# Autodesk Inventor assembly: SC8UU
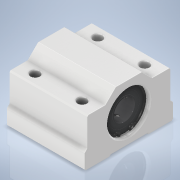
[picture p0: Inventor's stored thumbnail of the model, 180x180]
Saved by Autodesk Inventor 2020.2 (Build 242310000, 310)
## iProperties
Created: 2020-07-09
Part Number: SC8UU
Document SubType Name: Assembly
Designer: Artur Lenart
Author: Artur Lenart
## Documents named in this file (6)
- E:\Pliki\Inventor\Materiały\SC8UU\SC8UU.iam
- E:\Pliki\Inventor\Materiały\SC8UU\SC8 bearing ball.ipt
- E:\Pliki\Inventor\Materiały\SC8UU\SC8 bearing ext.ipt
- E:\Pliki\Inventor\Materiały\SC8UU\SC8 bearing int.ipt
- E:\Pliki\Inventor\Materiały\SC8UU\SC8UU body.ipt
- E:\Pliki\Inventor\Materiały\SC8UU\Seger.ipt
## Components (61 placed, 5 different names)
1. SC8 bearing ball:1 — Zestawiające:1, Styczny:1
2. SC8 bearing ext:1 — Zestawiające:57, Równoległe:1, Zestawiające:58, Równoległe:2
3. SC8 bearing int:1 — Zestawiające:1, Zestawiające:2, Zestawiające:3, Zestawiające:4, Zestawiające:5, Zestawiające:6, Zestawiające:7, Zestawiające:8, Zestawiające:9, Zestawiające:10, Zestawiające:11, Zestawiające:12, Zestawiające:13, Zestawiające:14, Zestawiające:15, Zestawiające:16, Zestawiające:17, Zestawiające:18, Zestawiające:19, Zestawiające:20, Zestawiające:21, Zestawiające:22, Zestawiające:23, Zestawiające:24, Zestawiające:25, Zestawiające:26, Zestawiające:27, Zestawiające:28, Zestawiające:29, Zestawiające:30, Zestawiające:31, Zestawiające:32, Zestawiające:33, Zestawiające:34, Zestawiające:35, Zestawiające:36, Zestawiające:37, Zestawiające:38, Zestawiające:39, Zestawiające:40, Zestawiające:41, Zestawiające:42, Zestawiające:43, Zestawiające:44, Zestawiające:45, Zestawiające:46, Zestawiające:47, Zestawiające:48, Zestawiające:49, Zestawiające:50, Zestawiające:51, Zestawiające:52, Zestawiające:53, Zestawiające:54, Zestawiające:55, Zestawiające:56, Zestawiające:57, Równoległe:1, Równoległe:4
4. SC8UU body:1 — Zestawiające:58, Równoległe:2, Zestawiające:59, Zestawiające:60, Zestawiające:61, Zestawiające:62
5. Seger:1 — Zestawiające:60, Równoległe:3, Równoległe:4, Zestawiające:61
6. Seger:2 — Zestawiające:59, Równoległe:3, Zestawiające:62
7. SC8 bearing ball:2 — Zestawiające:2, Styczny:2, Styczny:3
8. SC8 bearing ball:3 — Zestawiające:3, Styczny:3, Styczny:4
9. SC8 bearing ball:4 — Zestawiające:5, Styczny:4, Styczny:5
10. SC8 bearing ball:5 — Zestawiające:4, Styczny:5, Styczny:6
11. SC8 bearing ball:6 — Zestawiające:8, Styczny:7, Styczny:8
12. SC8 bearing ball:7 — Zestawiające:6, Styczny:8, Styczny:9
13. SC8 bearing ball:8 — Zestawiające:7, Styczny:6, Styczny:7
14. SC8 bearing ball:9 — Zestawiające:9, Styczny:1, Styczny:2
15. SC8 bearing ball:10 — Zestawiające:10, Styczny:9, Styczny:10
16. SC8 bearing ball:11 — Zestawiające:11, Styczny:10, Styczny:11
17. SC8 bearing ball:12 — Zestawiające:12, Styczny:11
18. SC8 bearing ball:13 — Zestawiające:13, Styczny:12
19. SC8 bearing ball:14 — Zestawiające:14, Styczny:12
20. SC8 bearing ball:15 — Zestawiające:16, Styczny:15, Styczny:16
21. SC8 bearing ball:16 — Zestawiające:20, Styczny:19, Styczny:20
22. SC8 bearing ball:17 — Zestawiające:19, Styczny:18, Styczny:19
23. SC8 bearing ball:18 — Zestawiające:21, Styczny:16, Styczny:17
24. SC8 bearing ball:19 — Zestawiające:18, Styczny:17, Styczny:18
25. SC8 bearing ball:20 — Zestawiające:17, Styczny:13, Styczny:14
26. SC8 bearing ball:21 — Zestawiające:28, Styczny:22
27. SC8 bearing ball:22 — Zestawiające:27, Styczny:21
28. SC8 bearing ball:23 — Zestawiające:26, Styczny:21, Styczny:23
29. SC8 bearing ball:24 — Zestawiające:25, Styczny:23, Styczny:24
30. SC8 bearing ball:25 — Zestawiające:23, Styczny:20
31. SC8 bearing ball:26 — Zestawiające:15, Styczny:13, Styczny:22
32. SC8 bearing ball:27 — Zestawiające:22, Styczny:14, Styczny:15
33. SC8 bearing ball:28 — Zestawiające:24, Styczny:24
34. SC8 bearing ball:29 — Zestawiające:42, Styczny:36
35. SC8 bearing ball:30 — Zestawiające:32, Styczny:27, Styczny:28
36. SC8 bearing ball:31 — Zestawiające:29, Styczny:25
37. SC8 bearing ball:32 — Zestawiające:31, Styczny:26, Styczny:27
38. SC8 bearing ball:33 — Zestawiające:33, Styczny:28, Styczny:29
39. SC8 bearing ball:34 — Zestawiające:37, Styczny:30, Styczny:31
40. SC8 bearing ball:35 — Zestawiające:36, Styczny:34, Styczny:35
41. SC8 bearing ball:36 — Zestawiające:39, Styczny:33, Styczny:34
42. SC8 bearing ball:37 — Zestawiające:35, Styczny:32, Styczny:36
43. SC8 bearing ball:38 — Zestawiające:30, Styczny:25, Styczny:26
44. SC8 bearing ball:39 — Zestawiające:38, Styczny:31, Styczny:32
45. SC8 bearing ball:40 — Zestawiające:40, Styczny:33
46. SC8 bearing ball:41 — Zestawiające:41, Styczny:35
47. SC8 bearing ball:42 — Zestawiające:34, Styczny:29, Styczny:30
48. SC8 bearing ball:43 — Zestawiające:46, Styczny:42
49. SC8 bearing ball:44 — Zestawiające:47, Styczny:40, Styczny:41
50. SC8 bearing ball:45 — Zestawiające:48, Styczny:39, Styczny:40
51. SC8 bearing ball:46 — Zestawiające:49, Styczny:41, Styczny:42
52. SC8 bearing ball:47 — Zestawiające:52, Styczny:38, Styczny:39
53. SC8 bearing ball:48 — Zestawiające:45, Styczny:44, Styczny:45
54. SC8 bearing ball:49 — Zestawiające:50, Styczny:37
55. SC8 bearing ball:50 — Zestawiające:53, Styczny:45, Styczny:46
56. SC8 bearing ball:51 — Zestawiające:55, Styczny:47, Styczny:48
57. SC8 bearing ball:52 — Zestawiające:44, Styczny:43, Styczny:44
58. SC8 bearing ball:53 — Zestawiające:54, Styczny:46, Styczny:47
59. SC8 bearing ball:54 — Zestawiające:56, Styczny:48
60. SC8 bearing ball:55 — Zestawiające:51, Styczny:37, Styczny:38
61. SC8 bearing ball:56 — Zestawiające:43, Styczny:43
## Relationships (114: Mate 62, Tangent 48, Flush 4)
- Zestawiające:1 [Mate]: SC8 bearing ball:1 ↔ SC8 bearing int:1
- Zestawiające:2 [Mate]: SC8 bearing int:1 ↔ SC8 bearing ball:2
- Zestawiające:3 [Mate]: SC8 bearing int:1 ↔ SC8 bearing ball:3
- Zestawiające:4 [Mate]: SC8 bearing int:1 ↔ SC8 bearing ball:5
- Zestawiające:5 [Mate]: SC8 bearing int:1 ↔ SC8 bearing ball:4
- Zestawiające:6 [Mate]: SC8 bearing int:1 ↔ SC8 bearing ball:7
- Zestawiające:7 [Mate]: SC8 bearing int:1 ↔ SC8 bearing ball:8
- Zestawiające:8 [Mate]: SC8 bearing int:1 ↔ SC8 bearing ball:6
- Zestawiające:9 [Mate]: SC8 bearing int:1 ↔ SC8 bearing ball:9
- Styczny:1 [Tangent]: SC8 bearing ball:1 ↔ SC8 bearing ball:9
- Styczny:2 [Tangent]: SC8 bearing ball:2 ↔ SC8 bearing ball:9
- Styczny:3 [Tangent]: SC8 bearing ball:2 ↔ SC8 bearing ball:3
- Styczny:4 [Tangent]: SC8 bearing ball:3 ↔ SC8 bearing ball:4
- Styczny:5 [Tangent]: SC8 bearing ball:4 ↔ SC8 bearing ball:5
- Styczny:6 [Tangent]: SC8 bearing ball:5 ↔ SC8 bearing ball:8
- Styczny:7 [Tangent]: SC8 bearing ball:6 ↔ SC8 bearing ball:8
- Styczny:8 [Tangent]: SC8 bearing ball:6 ↔ SC8 bearing ball:7
- Zestawiające:10 [Mate]: SC8 bearing int:1 ↔ SC8 bearing ball:10
- Zestawiające:11 [Mate]: SC8 bearing int:1 ↔ SC8 bearing ball:11
- Zestawiające:12 [Mate]: SC8 bearing int:1 ↔ SC8 bearing ball:12
- Styczny:9 [Tangent]: SC8 bearing ball:7 ↔ SC8 bearing ball:10
- Styczny:10 [Tangent]: SC8 bearing ball:10 ↔ SC8 bearing ball:11
- Styczny:11 [Tangent]: SC8 bearing ball:11 ↔ SC8 bearing ball:12
- Zestawiające:13 [Mate]: SC8 bearing int:1 ↔ SC8 bearing ball:13
- Zestawiające:14 [Mate]: SC8 bearing int:1 ↔ SC8 bearing ball:14
- Styczny:12 [Tangent]: SC8 bearing ball:13 ↔ SC8 bearing ball:14
- Zestawiające:15 [Mate]: SC8 bearing int:1 ↔ SC8 bearing ball:26
- Zestawiające:16 [Mate]: SC8 bearing int:1 ↔ SC8 bearing ball:15
- Zestawiające:17 [Mate]: SC8 bearing int:1 ↔ SC8 bearing ball:20
- Zestawiające:18 [Mate]: SC8 bearing int:1 ↔ SC8 bearing ball:19
- Zestawiające:19 [Mate]: SC8 bearing int:1 ↔ SC8 bearing ball:17
- Zestawiające:20 [Mate]: SC8 bearing int:1 ↔ SC8 bearing ball:16
- Zestawiające:21 [Mate]: SC8 bearing int:1 ↔ SC8 bearing ball:18
- Zestawiające:22 [Mate]: SC8 bearing int:1 ↔ SC8 bearing ball:27
- Zestawiające:23 [Mate]: SC8 bearing int:1 ↔ SC8 bearing ball:25
- Styczny:13 [Tangent]: SC8 bearing ball:20 ↔ SC8 bearing ball:26
- Styczny:14 [Tangent]: SC8 bearing ball:20 ↔ SC8 bearing ball:27
- Styczny:15 [Tangent]: SC8 bearing ball:15 ↔ SC8 bearing ball:27
- Styczny:16 [Tangent]: SC8 bearing ball:15 ↔ SC8 bearing ball:18
- Styczny:17 [Tangent]: SC8 bearing ball:18 ↔ SC8 bearing ball:19
- Styczny:18 [Tangent]: SC8 bearing ball:17 ↔ SC8 bearing ball:19
- Styczny:19 [Tangent]: SC8 bearing ball:16 ↔ SC8 bearing ball:17
- Styczny:20 [Tangent]: SC8 bearing ball:16 ↔ SC8 bearing ball:25
- Zestawiające:24 [Mate]: SC8 bearing int:1 ↔ SC8 bearing ball:28
- Zestawiające:25 [Mate]: SC8 bearing int:1 ↔ SC8 bearing ball:24
- Zestawiające:26 [Mate]: SC8 bearing int:1 ↔ SC8 bearing ball:23
- Zestawiające:27 [Mate]: SC8 bearing int:1 ↔ SC8 bearing ball:22
- Zestawiające:28 [Mate]: SC8 bearing int:1 ↔ SC8 bearing ball:21
- Styczny:21 [Tangent]: SC8 bearing ball:22 ↔ SC8 bearing ball:23
- Styczny:22 [Tangent]: SC8 bearing ball:21 ↔ SC8 bearing ball:26
- Styczny:23 [Tangent]: SC8 bearing ball:23 ↔ SC8 bearing ball:24
- Styczny:24 [Tangent]: SC8 bearing ball:24 ↔ SC8 bearing ball:28
- Zestawiające:29 [Mate]: SC8 bearing int:1 ↔ SC8 bearing ball:31
- Zestawiające:30 [Mate]: SC8 bearing int:1 ↔ SC8 bearing ball:38
- Zestawiające:31 [Mate]: SC8 bearing int:1 ↔ SC8 bearing ball:32
- Zestawiające:32 [Mate]: SC8 bearing int:1 ↔ SC8 bearing ball:30
- Zestawiające:33 [Mate]: SC8 bearing int:1 ↔ SC8 bearing ball:33
- Zestawiające:34 [Mate]: SC8 bearing int:1 ↔ SC8 bearing ball:42
- Zestawiające:35 [Mate]: SC8 bearing int:1 ↔ SC8 bearing ball:37
- Zestawiające:36 [Mate]: SC8 bearing int:1 ↔ SC8 bearing ball:35
- Zestawiające:37 [Mate]: SC8 bearing int:1 ↔ SC8 bearing ball:34
- Zestawiające:38 [Mate]: SC8 bearing int:1 ↔ SC8 bearing ball:39
- Zestawiające:39 [Mate]: SC8 bearing int:1 ↔ SC8 bearing ball:36
- Zestawiające:40 [Mate]: SC8 bearing int:1 ↔ SC8 bearing ball:40
- Styczny:25 [Tangent]: SC8 bearing ball:31 ↔ SC8 bearing ball:38
- Styczny:26 [Tangent]: SC8 bearing ball:32 ↔ SC8 bearing ball:38
- Styczny:27 [Tangent]: SC8 bearing ball:30 ↔ SC8 bearing ball:32
- Styczny:28 [Tangent]: SC8 bearing ball:30 ↔ SC8 bearing ball:33
- Styczny:29 [Tangent]: SC8 bearing ball:33 ↔ SC8 bearing ball:42
- Styczny:30 [Tangent]: SC8 bearing ball:34 ↔ SC8 bearing ball:42
- Styczny:31 [Tangent]: SC8 bearing ball:34 ↔ SC8 bearing ball:39
- Styczny:32 [Tangent]: SC8 bearing ball:37 ↔ SC8 bearing ball:39
- Styczny:33 [Tangent]: SC8 bearing ball:36 ↔ SC8 bearing ball:40
- Styczny:34 [Tangent]: SC8 bearing ball:35 ↔ SC8 bearing ball:36
- Zestawiające:41 [Mate]: SC8 bearing int:1 ↔ SC8 bearing ball:41
- Styczny:35 [Tangent]: SC8 bearing ball:35 ↔ SC8 bearing ball:41
- Zestawiające:42 [Mate]: SC8 bearing int:1 ↔ SC8 bearing ball:29
- Styczny:36 [Tangent]: SC8 bearing ball:29 ↔ SC8 bearing ball:37
- Zestawiające:43 [Mate]: SC8 bearing int:1 ↔ SC8 bearing ball:56
- Zestawiające:44 [Mate]: SC8 bearing int:1 ↔ SC8 bearing ball:52
- Zestawiające:45 [Mate]: SC8 bearing int:1 ↔ SC8 bearing ball:48
- Zestawiające:46 [Mate]: SC8 bearing int:1 ↔ SC8 bearing ball:43
- Zestawiające:47 [Mate]: SC8 bearing int:1 ↔ SC8 bearing ball:44
- Zestawiające:48 [Mate]: SC8 bearing int:1 ↔ SC8 bearing ball:45
- Zestawiające:49 [Mate]: SC8 bearing int:1 ↔ SC8 bearing ball:46
- Zestawiające:50 [Mate]: SC8 bearing int:1 ↔ SC8 bearing ball:49
- Zestawiające:51 [Mate]: SC8 bearing int:1 ↔ SC8 bearing ball:55
- Zestawiające:52 [Mate]: SC8 bearing int:1 ↔ SC8 bearing ball:47
- Styczny:37 [Tangent]: SC8 bearing ball:49 ↔ SC8 bearing ball:55
- Styczny:38 [Tangent]: SC8 bearing ball:47 ↔ SC8 bearing ball:55
- Styczny:39 [Tangent]: SC8 bearing ball:45 ↔ SC8 bearing ball:47
- Styczny:40 [Tangent]: SC8 bearing ball:44 ↔ SC8 bearing ball:45
- Styczny:41 [Tangent]: SC8 bearing ball:44 ↔ SC8 bearing ball:46
- Styczny:42 [Tangent]: SC8 bearing ball:43 ↔ SC8 bearing ball:46
- Styczny:43 [Tangent]: SC8 bearing ball:52 ↔ SC8 bearing ball:56
- Styczny:44 [Tangent]: SC8 bearing ball:48 ↔ SC8 bearing ball:52
- Zestawiające:53 [Mate]: SC8 bearing int:1 ↔ SC8 bearing ball:50
- Zestawiające:54 [Mate]: SC8 bearing int:1 ↔ SC8 bearing ball:53
- Zestawiające:55 [Mate]: SC8 bearing int:1 ↔ SC8 bearing ball:51
- Styczny:45 [Tangent]: SC8 bearing ball:48 ↔ SC8 bearing ball:50
- Styczny:46 [Tangent]: SC8 bearing ball:50 ↔ SC8 bearing ball:53
- Styczny:47 [Tangent]: SC8 bearing ball:51 ↔ SC8 bearing ball:53
- Zestawiające:56 [Mate]: SC8 bearing int:1 ↔ SC8 bearing ball:54
- Styczny:48 [Tangent]: SC8 bearing ball:51 ↔ SC8 bearing ball:54
- Zestawiające:57 [Mate]: SC8 bearing ext:1 ↔ SC8 bearing int:1
- Równoległe:1 [Flush]: SC8 bearing ext:1 ↔ SC8 bearing int:1
- Zestawiające:58 [Mate]: SC8 bearing ext:1 ↔ SC8UU body:1
- Równoległe:2 [Flush] (-2 mm): SC8 bearing ext:1 ↔ SC8UU body:1
- Zestawiające:59 [Mate]: SC8UU body:1 ↔ Seger:2
- Zestawiające:60 [Mate]: SC8UU body:1 ↔ Seger:1
- Równoległe:3 [Flush]: Seger:1 ↔ Seger:2
- Równoległe:4 [Flush]: SC8 bearing int:1 ↔ Seger:1
- Zestawiające:61 [Mate]: SC8UU body:1 ↔ Seger:1
- Zestawiające:62 [Mate]: SC8UU body:1 ↔ Seger:2
